# Autodesk Inventor assembly: LMbot V3
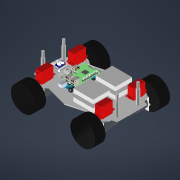
[picture p0: Inventor's stored thumbnail of the model, 180x180]
Saved by Autodesk Inventor 2021 (Build 250183000, 183)
## iProperties
Company: none
Created: 2021-01-23
Part Number: LMbot V3
Description: CATIA V5 STEP Exchange
Document SubType Name: Assembly
Designer: Ashiqrahman
Authority: none
Sending System: CATIA V5 STEP AP203
Preprocessor: CATIA Version 5 Release 20 GA (IN-10)
Title: E:\ENGINEERING\tomohawk\Assembly\LMbot V3\LMbot V3.stp
Author: none
## Documents named in this file (12)
- D:\Projects\P_Line Marking Bot\Design\LMbot V3\LMbot V3.iam
- D:\Projects\P_Line Marking Bot\Design\LMbot V3\chasis.ipt
- D:\Projects\P_Line Marking Bot\Design\LMbot V3\MG-958 servo.iam
- D:\Projects\P_Line Marking Bot\Design\LMbot V3\knucle.ipt
- D:\Projects\P_Line Marking Bot\Design\LMbot V3\JGB37-520.iam
- D:\Projects\P_Line Marking Bot\Design\LMbot V3\wheel .ipt
- D:\Projects\P_Line Marking Bot\Design\LMbot V3\Part1.ipt
- D:\Projects\A_Electronics CAD model\Rasberry pi\Arduino Mega ATmega 2560.iam
- D:\Projects\P_Line Marking Bot\Design\LMbot V3\RaspberryPi.iam
- D:\Projects\A_Electronics CAD model\ublox-gps-1.snapshot.1\gps\parts\GPS_ublox_board.ipt
- D:\Projects\A_Electronics CAD model\mpu-9250-9dof-imu-1.snapshot.4\MPU-9250.iam
- C:\Users\Ashiqrahman\Documents\motor driver.ipt
## Components (26 placed, 15 different names)
1. chasis — Mate:1, Mate:2, Mate:3, Mate:4, Mate:5, Mate:7, Mate:8, Mate:9, Mate:10, Mate:11, Mate:14, Mate:16, Mate:17, Mate:36, Flush:5, Mate:37, Flush:6, Mate:38, Flush:7, Flush:8, Flush:9, Flush:10, Mate:40, Mate:41, Mate:42, Flush:13, Flush:19, Mate:43, Mate:44
2. MG-958 servo.1 [sub-assembly] — Flush:1, Mate:15, Mate:16, Mate:17
3. knucle.2 — Mate:14, Mate:15, Mate:20, Mate:21
4. JGB37-520.1 [sub-assembly] — Mate:24, Mate:25, Mate:28, Mate:30, Mate:46
5. wheel .1 — Mate:26, Mate:32, Flush:3
6. Part1.3 — Flush:14, Flush:19, Mate:43, Mate:44
7. MG-958 servo:2 [sub-assembly] — Mate:1, Mate:2, Flush:2, Mate:6
8. MG-958 servo:3 [sub-assembly] — Mate:3, Flush:1, Mate:42
9. MG-958 servo:4 [sub-assembly] — Mate:4, Mate:5, Flush:2, Mate:39
10. knucle:2 — Mate:8, Mate:9, Mate:24, Mate:25
11. knucle:3 — Mate:6, Mate:7, Mate:18, Mate:19
12. knucle:4 — Mate:10, Mate:11, Mate:22, Mate:23
13. JGB37-520:2 [sub-assembly] — Mate:22, Mate:23, Mate:34, Mate:35, Mate:45
14. JGB37-520:3 [sub-assembly] — Mate:20, Mate:21, Mate:26, Mate:32, Mate:46
15. JGB37-520:4 [sub-assembly] — Mate:18, Mate:19, Mate:27, Mate:33, Mate:45
16. wheel :2 — Mate:27, Mate:33, Flush:3
17. wheel :3 — Mate:34, Mate:35, Flush:4
18. wheel :4 — Mate:28, Mate:30, Flush:4
19. Arduino Mega ATmega 2560:1 [sub-assembly] — Mate:36, Flush:5, Flush:10, Flush:11
20. RaspberryPi:1 [sub-assembly] — Mate:37, Flush:6, Flush:11
21. GPS_ublox_board:1 — Mate:38, Flush:7
22. MPU-9250:1 [sub-assembly] — Flush:8, Flush:9, Mate:39
23. motor driver:1 — Flush:16, Flush:17, Flush:20
24. motor driver:2 — Mate:40, Flush:12, Flush:15, Flush:18, Flush:21
25. motor driver:3 — Mate:41, Flush:12, Flush:13, Flush:14, Flush:15
26. motor driver:4 — Flush:16, Flush:17, Flush:18, Flush:20, Flush:21
## Relationships (63: Mate 42, Flush 21)
- Mate:1: chasis ↔ MG-958 servo:2
- Mate:2: chasis ↔ MG-958 servo:2
- Mate:3: chasis ↔ MG-958 servo:3
- Mate:4: chasis ↔ MG-958 servo:4
- Mate:5: chasis ↔ MG-958 servo:4
- Flush:1: MG-958 servo.1 ↔ MG-958 servo:3
- Flush:2: MG-958 servo:2 ↔ MG-958 servo:4
- Mate:6: MG-958 servo:2 ↔ knucle:3
- Mate:7: chasis ↔ knucle:3
- Mate:8: chasis ↔ knucle:2
- Mate:9: chasis ↔ knucle:2
- Mate:10: chasis ↔ knucle:4
- Mate:11: chasis ↔ knucle:4
- Mate:14: chasis ↔ knucle.2
- Mate:15: MG-958 servo.1 ↔ knucle.2
- Mate:16: chasis ↔ MG-958 servo.1
- Mate:17: chasis ↔ MG-958 servo.1
- Mate:18: knucle:3 ↔ JGB37-520:4
- Mate:19: knucle:3 ↔ JGB37-520:4
- Mate:20: knucle.2 ↔ JGB37-520:3
- Mate:21: knucle.2 ↔ JGB37-520:3
- Mate:22: knucle:4 ↔ JGB37-520:2
- Mate:23: knucle:4 ↔ JGB37-520:2
- Mate:24: JGB37-520.1 ↔ knucle:2
- Mate:25: JGB37-520.1 ↔ knucle:2
- Mate:26: wheel .1 ↔ JGB37-520:3
- Mate:27: JGB37-520:4 ↔ wheel :2
- Mate:28: JGB37-520.1 ↔ wheel :4
- Mate:30 (-5 mm): JGB37-520.1 ↔ wheel :4
- Mate:32 (5 mm): wheel .1 ↔ JGB37-520:3
- Mate:33 (-5 mm): JGB37-520:4 ↔ wheel :2
- Flush:3: wheel .1 ↔ wheel :2
- Mate:34: JGB37-520:2 ↔ wheel :3
- Mate:35 (-5 mm): JGB37-520:2 ↔ wheel :3
- Flush:4: wheel :3 ↔ wheel :4
- Mate:36: chasis ↔ Arduino Mega ATmega 2560:1
- Flush:5 (75 mm): chasis ↔ Arduino Mega ATmega 2560:1
- Mate:37 (20 mm): chasis ↔ RaspberryPi:1
- Flush:6 (75 mm): chasis ↔ RaspberryPi:1
- Mate:38: chasis ↔ GPS_ublox_board:1
- Flush:7: chasis ↔ GPS_ublox_board:1
- Flush:8 (-20 mm): chasis ↔ MPU-9250:1
- Flush:9 (30 mm): chasis ↔ MPU-9250:1
- Mate:39 (20 mm): MG-958 servo:4 ↔ MPU-9250:1
- Flush:10 (-10 mm): chasis ↔ Arduino Mega ATmega 2560:1
- Flush:11: Arduino Mega ATmega 2560:1 ↔ RaspberryPi:1
- Mate:40: chasis ↔ motor driver:2
- Mate:41: chasis ↔ motor driver:3
- Mate:42: chasis ↔ MG-958 servo:3
- Flush:12: motor driver:2 ↔ motor driver:3
- Flush:13 (65 mm): chasis ↔ motor driver:3
- Flush:14 (60 mm): Part1.3 ↔ motor driver:3
- Flush:15 (-75 mm): motor driver:2 ↔ motor driver:3
- Flush:16: motor driver:1 ↔ motor driver:4
- Flush:17: motor driver:1 ↔ motor driver:4
- Flush:18: motor driver:2 ↔ motor driver:4
- Flush:19: chasis ↔ Part1.3
- Mate:43: chasis ↔ Part1.3
- Mate:44: chasis ↔ Part1.3
- Flush:20 (-75 mm): motor driver:1 ↔ motor driver:4
- Flush:21: motor driver:2 ↔ motor driver:4
- Mate:45: JGB37-520:2 ↔ JGB37-520:4
- Mate:46: JGB37-520.1 ↔ JGB37-520:3
